# Autodesk Inventor assembly: Assembly146-01
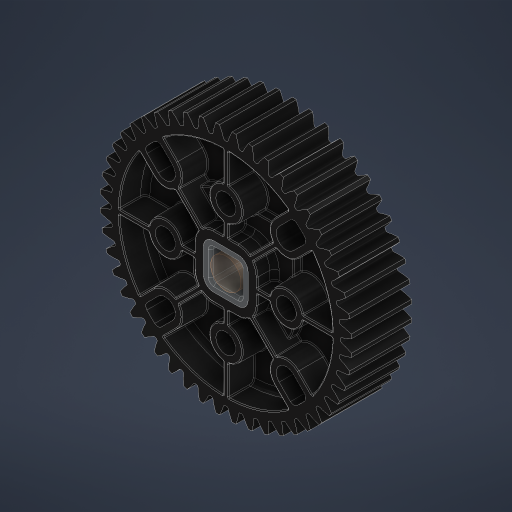
[picture p0: Inventor's stored thumbnail of the model, 512x512]
Saved by Autodesk Inventor 2024 (Build 280153000, 153)
## iProperties
Created: 2022-08-02
Part Number: Assembly146-01
Document SubType Name: Assembly
Designer: ylu12
Author: ylu12
## Documents named in this file (3)
- D:\vex_robotics\hardware\cad\VEX-CAD-Inventor-1.41\Motion\Gears\HS Gear\HS 48T Gear, No Insert.iam
- D:\vex_robotics\hardware\cad\VEX-CAD-Inventor-1.41\Motion\Gears\Reference Files\HS 48T Gear, No Insert.ipt
- D:\vex_robotics\hardware\cad\VEX-CAD-Inventor-1.41\Motion\Gears\HS Gear.iam
## Components (1 placed, 1 different names)
1. 48T — Flush:6, Mate:11, Mate:12
## Relationships (3: Mate 2, Flush 1)
- Flush:6: 48T
- Mate:11: 48T
- Mate:12: 48T
